# Autodesk Inventor assembly: MKS TFT
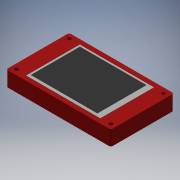
[picture p0: Inventor's stored thumbnail of the model, 180x180]
Saved by Autodesk Inventor 2018.2 (Build 222227000, 227)
## iProperties
Created: 2018-04-02
Part Number: MKS TFT
Material: Generisch
Document SubType Name: Assembly
Designer: Till
Author: Till
## Documents named in this file (3)
- C:\Users\Till\Dropbox\Ultibox\ultibox\cad\MKS TFT.iam
- C:\Users\Till\Dropbox\Ultibox\ultibox\cad\MKS TFT32.ipt
- C:\Users\Till\Dropbox\Ultibox\ultibox\cad\front_case.ipt
## Components (2 placed, 2 different names)
1. MKS TFT32:1 — Fluchtend:1
2. front_case:1 — Fluchtend:1
## Relationships (1: Flush 1)
- Fluchtend:1 [Flush]: MKS TFT32:1 ↔ front_case:1
